# Autodesk Inventor assembly: Hopper Nut Trap assy
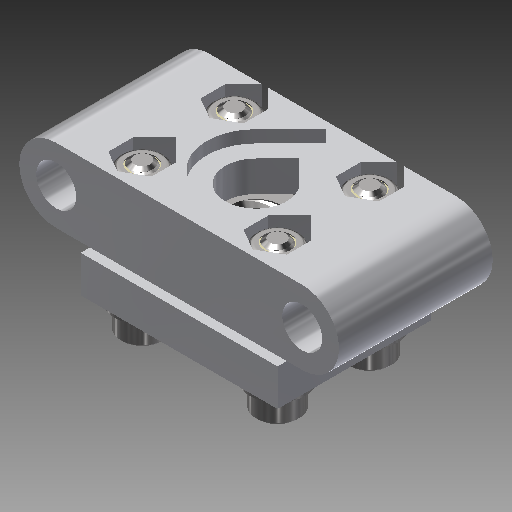
[picture p0: Inventor's stored thumbnail of the model, 512x512]
Saved by Autodesk Inventor 2018 (Build 220112000, 112)
## iProperties
Created: 2017-09-27
Part Number: Hopper Nut Trap assy
Document SubType Name: Assembly
Designer: Gabriel Smolnycki
Author: Gabriel Smolnycki
## Documents named in this file (7)
- E:\planb\mechanics\Subassemblies\Hopper Nut Trap assy.iam
- E:\planb\mechanics\Hopper\Hopper Nut Trap.ipt
- E:\planb\mechanics\Hopper\Hopper Nut Trap Holder.ipt
- E:\planb\mechanics\Hardware\M8 SS Nut.ipt
- E:\planb\mechanics\Hardware\M4x20 SS SHCS.ipt
- E:\planb\mechanics\Hardware\M4 SS Washer.ipt
- E:\planb\mechanics\Hardware\M4 SS Locknut.ipt
## Components (15 placed, 6 different names)
1. Hopper Nut Trap:1 — Insert:1, Mate:1, Flush:1, Insert:3, Mate:2, Insert:8, Mate:3, Insert:9, Mate:4, Insert:10, Mate:5
2. Hopper Nut Trap Holder:1 — Insert:2, Flush:1, Insert:4, Insert:5, Insert:6, Insert:7
3. M8 SS Nut:1 — Insert:1, Mate:1, Insert:2
4. M4x20 SS SHCS:1 — Insert:13
5. M4x20 SS SHCS:2 — Insert:14
6. M4x20 SS SHCS:3 — Insert:12
7. M4x20 SS SHCS:4 — Insert:11
8. M4 SS Washer:1 — Insert:7, Insert:11
9. M4 SS Washer:2 — Insert:6, Insert:13
10. M4 SS Washer:3 — Insert:5, Insert:14
11. M4 SS Washer:4 — Insert:4, Insert:12
12. M4 SS Locknut:1 — Insert:8, Mate:3
13. M4 SS Locknut:2 — Insert:9, Mate:4
14. M4 SS Locknut:3 — Insert:10, Mate:5
15. M4 SS Locknut:4 — Insert:3, Mate:2
## Relationships (20: Insert 14, Mate 5, Flush 1)
- Insert:1: Hopper Nut Trap:1 ↔ M8 SS Nut:1
- Mate:1: Hopper Nut Trap:1 ↔ M8 SS Nut:1
- Insert:2: Hopper Nut Trap Holder:1 ↔ M8 SS Nut:1
- Flush:1: Hopper Nut Trap:1 ↔ Hopper Nut Trap Holder:1
- Insert:3: Hopper Nut Trap:1 ↔ M4 SS Locknut:4
- Mate:2: Hopper Nut Trap:1 ↔ M4 SS Locknut:4
- Insert:4: Hopper Nut Trap Holder:1 ↔ M4 SS Washer:4
- Insert:5: Hopper Nut Trap Holder:1 ↔ M4 SS Washer:3
- Insert:6: Hopper Nut Trap Holder:1 ↔ M4 SS Washer:2
- Insert:7: Hopper Nut Trap Holder:1 ↔ M4 SS Washer:1
- Insert:8: Hopper Nut Trap:1 ↔ M4 SS Locknut:1
- Mate:3: Hopper Nut Trap:1 ↔ M4 SS Locknut:1
- Insert:9: Hopper Nut Trap:1 ↔ M4 SS Locknut:2
- Mate:4: Hopper Nut Trap:1 ↔ M4 SS Locknut:2
- Insert:10: Hopper Nut Trap:1 ↔ M4 SS Locknut:3
- Mate:5: Hopper Nut Trap:1 ↔ M4 SS Locknut:3
- Insert:11: M4x20 SS SHCS:4 ↔ M4 SS Washer:1
- Insert:12: M4x20 SS SHCS:3 ↔ M4 SS Washer:4
- Insert:13: M4x20 SS SHCS:1 ↔ M4 SS Washer:2
- Insert:14: M4x20 SS SHCS:2 ↔ M4 SS Washer:3
